# Autodesk Inventor assembly: #Climber
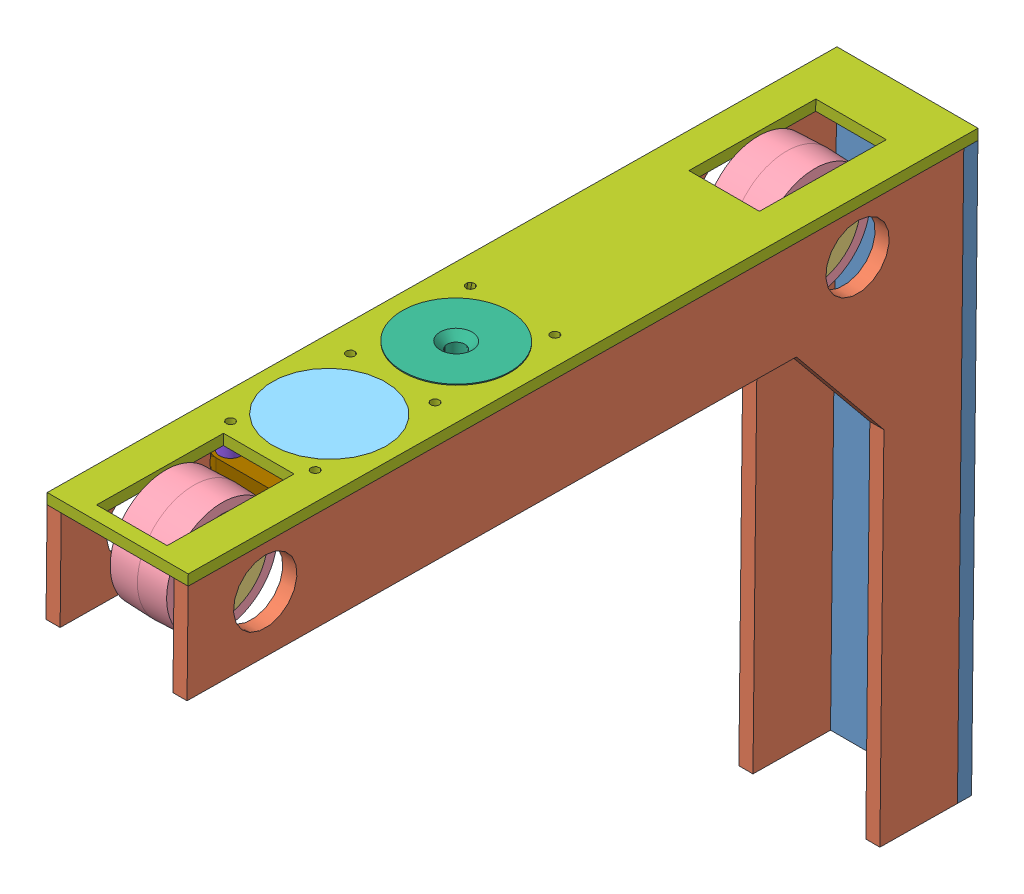
[picture p0: shaded view drawn from the shape stored in the file]
Saved by Autodesk Inventor 2026.1 (Build 301233020, 233B)
## iProperties
Created: 2026-03-19
Part Number: #Climber
Document SubType Name: Assembly
Designer: Owen L
Mass: 1648.82 g
Surface Area: 2308.56 cm^2
Volume: 580.188 cm^3
Density: 2.84187 g/cm^3
Author: Owen L
## Documents named in this file (9)
- C:\Users\Owen\Documents\GitHub\2026-Robot-Mechanical\Climb\#Climber.iam
- C:\Users\Owen\Documents\GitHub\2026-Robot-Mechanical\Climb\PLATE,FRONT.ipt
- C:\Users\Owen\Documents\GitHub\2026-Robot-Mechanical\Climb\PLATE,BOTTOM.ipt
- C:\Users\Owen\Documents\GitHub\2026-Robot-Mechanical\Climb\PLATE,GUSSET.ipt
- C:\Users\Owen\Documents\GitHub\2026-Robot-Mechanical\Climb\am-3155 2in 500Hex Stealth Wheel REV2.ipt
- C:\Users\Owen\Documents\GitHub\2026-Robot-Mechanical\Climb\BIG-MAGNET.ipt
- C:\Users\Owen\Documents\GitHub\2026-Robot-Mechanical\Climb\SMALL-MAGNET.ipt
- C:\Users\Owen\Documents\GitHub\2026-Robot-Mechanical\Climb\PLATE,MAGNET-MOUNT.ipt
- C:\Users\Owen\Documents\GitHub\2026-Robot-Mechanical\Climb\SPACER,MAGNET-PLATE.ipt
## Components (15 placed, 8 different names)
1. PLATE,FRONT:1 — Mate:1, Mate:2, Mate:3, Mate:8, Mate:10, Insert:1, Flush:1, Mate:13, Insert:8, Insert:9
2. PLATE,BOTTOM:1 — Mate:1, Mate:2, Mate:3, Mate:7, Mate:9
3. PLATE,GUSSET:1 — Mate:7, Mate:8, Mate:11
4. PLATE,GUSSET:2 — Mate:9, Mate:10, Mate:12
5. am-3155 2in 500Hex Stealth Wheel REV2:1 — Mate:12
6. am-3155 2in 500Hex Stealth Wheel REV2:2 — Mate:11
7. BIG-MAGNET:1 — Insert:1
8. SMALL-MAGNET:1 — Flush:1, Mate:13
9. PLATE,MAGNET-MOUNT:1 — Insert:2, Insert:3, Insert:4, Insert:5, Insert:6, Insert:7
10. SPACER,MAGNET-PLATE:1 — Insert:2, Insert:8
11. SPACER,MAGNET-PLATE:2 — Insert:3
12. SPACER,MAGNET-PLATE:3 — Insert:6, Insert:9
13. SPACER,MAGNET-PLATE:4 — Insert:7
14. SPACER,MAGNET-PLATE:5 — Insert:4
15. SPACER,MAGNET-PLATE:6 — Insert:5
## Relationships (20: Mate 10, Insert 9, Flush 1)
- Mate:1: PLATE,FRONT:1 ↔ PLATE,BOTTOM:1
- Mate:2: PLATE,FRONT:1 ↔ PLATE,BOTTOM:1
- Mate:3: PLATE,FRONT:1 ↔ PLATE,BOTTOM:1
- Mate:7: PLATE,BOTTOM:1 ↔ PLATE,GUSSET:1
- Mate:8: PLATE,FRONT:1 ↔ PLATE,GUSSET:1
- Mate:9: PLATE,BOTTOM:1 ↔ PLATE,GUSSET:2
- Mate:10: PLATE,FRONT:1 ↔ PLATE,GUSSET:2
- Mate:11: PLATE,GUSSET:1 ↔ am-3155 2in 500Hex Stealth Wheel REV2:2
- Mate:12: PLATE,GUSSET:2 ↔ am-3155 2in 500Hex Stealth Wheel REV2:1
- Insert:1: PLATE,FRONT:1 ↔ BIG-MAGNET:1
- Flush:1 (-6.3627 mm): PLATE,FRONT:1 ↔ SMALL-MAGNET:1
- Mate:13: PLATE,FRONT:1 ↔ SMALL-MAGNET:1
- Insert:2: PLATE,MAGNET-MOUNT:1 ↔ SPACER,MAGNET-PLATE:1
- Insert:3: PLATE,MAGNET-MOUNT:1 ↔ SPACER,MAGNET-PLATE:2
- Insert:4: PLATE,MAGNET-MOUNT:1 ↔ SPACER,MAGNET-PLATE:5
- Insert:5: PLATE,MAGNET-MOUNT:1 ↔ SPACER,MAGNET-PLATE:6
- Insert:6: PLATE,MAGNET-MOUNT:1 ↔ SPACER,MAGNET-PLATE:3
- Insert:7: PLATE,MAGNET-MOUNT:1 ↔ SPACER,MAGNET-PLATE:4
- Insert:8: PLATE,FRONT:1 ↔ SPACER,MAGNET-PLATE:1
- Insert:9: PLATE,FRONT:1 ↔ SPACER,MAGNET-PLATE:3
